# Autodesk Inventor assembly: Tread Sprocket Assembly
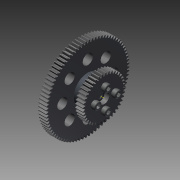
[picture p0: Inventor's stored thumbnail of the model, 180x180]
Saved by Autodesk Inventor 2015 (Build 190159000, 159)
## iProperties
Created: 2015-09-28
Part Number: Tread Sprocket Assembly
Document SubType Name: Assembly
Designer: Jing-Chen
Author: Jing-Chen
## Documents named in this file (5)
- C:\Users\Jing-Chen\Desktop\Bionic Hybrids 2016\Bionic-Hybrids\CAD\Drivetrain\Sub-Assemblies\Tread Sprocket Assembly.iam
- C:\Users\Jing-Chen\Desktop\Bionic Hybrids 2016\Bionic-Hybrids\Stock\Gear-40 tooth - 731901.ipt
- C:\Users\Jing-Chen\Desktop\Bionic Hybrids 2016\Bionic-Hybrids\CAD\Drivetrain\Modified Parts\Axle Hub - non-locking.ipt
- C:\Users\Jing-Chen\Desktop\Bionic Hybrids 2016\Bionic-Hybrids\CAD\Drivetrain\Modified Parts\1-inch Screw.ipt
- C:\Users\Jing-Chen\Desktop\Bionic Hybrids 2016\Bionic-Hybrids\Stock\Gear-80 tooth - 731901.ipt
## Components (8 placed, 4 different names)
1. Gear-40 tooth - 731901:1 — Mate:13, Mate:14, Mate:15, Mate:18, Mate:19, Mate:20, Mate:21
2. Axle Hub - non-locking:1 — Mate:29
3. Axle Hub - non-locking:2 — Mate:25, Mate:26, Mate:30
4. 1-inch Screw:1
5. 1-inch Screw:2 — Mate:25, Mate:27
6. 1-inch Screw:3 — Mate:19, Mate:21, Mate:26, Mate:28
7. 1-inch Screw:4 — Mate:18, Mate:20
8. Gear-80 tooth - 731901:1 — Mate:27, Mate:28, Mate:29, Mate:30
## Relationships (20: Mate 20)
- [Mate]: Gear-40 tooth - 731901:1 ↔ Axle Hub - non-locking:1
- [Mate]: Gear-40 tooth - 731901:1 ↔ Axle Hub - non-locking:1
- [Mate]: Gear-40 tooth - 731901:1 ↔ Axle Hub - non-locking:1
- [Mate]: Gear-40 tooth - 731901:1 ↔ 1-inch Screw:1
- [Mate]: Gear-40 tooth - 731901:1 ↔ 1-inch Screw:2
- [Mate]: Gear-40 tooth - 731901:1 ↔ 1-inch Screw:2
- [Mate]: Gear-40 tooth - 731901:1 ↔ 1-inch Screw:1
- Mate:13: Gear-40 tooth - 731901:1
- Mate:14: Gear-40 tooth - 731901:1
- Mate:15: Gear-40 tooth - 731901:1
- Mate:18: Gear-40 tooth - 731901:1 ↔ 1-inch Screw:4
- Mate:19: Gear-40 tooth - 731901:1 ↔ 1-inch Screw:3
- Mate:20: Gear-40 tooth - 731901:1 ↔ 1-inch Screw:4
- Mate:21: Gear-40 tooth - 731901:1 ↔ 1-inch Screw:3
- Mate:25: Axle Hub - non-locking:2 ↔ 1-inch Screw:2
- Mate:26: Axle Hub - non-locking:2 ↔ 1-inch Screw:3
- Mate:27: 1-inch Screw:2 ↔ Gear-80 tooth - 731901:1
- Mate:28: 1-inch Screw:3 ↔ Gear-80 tooth - 731901:1
- Mate:29: Axle Hub - non-locking:1 ↔ Gear-80 tooth - 731901:1
- Mate:30: Axle Hub - non-locking:2 ↔ Gear-80 tooth - 731901:1
